# Autodesk Inventor assembly: ASY MSC 800 gills
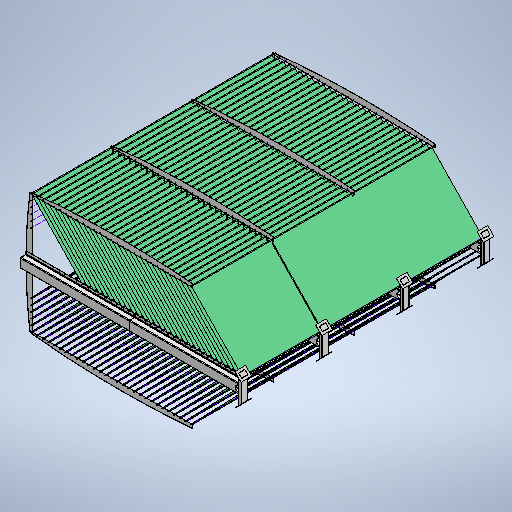
[picture p0: Inventor's stored thumbnail of the model, 512x512]
Saved by Autodesk Inventor 2025 (Build 290162010, 162A)
## iProperties
Created: 2024-08-31
Part Number: ASY MSC 800 gills
Document SubType Name: Assembly
Designer: pokla
Stock Number: ASY МОО 800 Жабры
Mass: 469810 g
Surface Area: 1.86943e+06 cm^2
Volume: 67870.7 cm^3
Density: 6.92212 g/cm^3
Author: pokla
## Documents named in this file (19)
- C:\Users\pokla\Documents\Inventor\Отстойник осветлитель\Manturovo_Se-clar-Gleb\ASY MSC 800 gills.iam
- C:\Users\pokla\Documents\Inventor\Отстойник осветлитель\Manturovo_Se-clar-Gleb\MSC 804 sheet gills.ipt
- C:\Users\pokla\Documents\Inventor\Отстойник осветлитель\Manturovo_Se-clar-Gleb\MSC 810 pillar gills.ipt
- C:\Users\pokla\Documents\Inventor\Отстойник осветлитель\Manturovo_Se-clar-Gleb\MSC 805 sheet gills.ipt
- C:\Users\pokla\Documents\Inventor\Отстойник осветлитель\Manturovo_Se-clar-Gleb\MSC 806 sheet gills.ipt
- C:\Users\pokla\Documents\Inventor\Отстойник осветлитель\Manturovo_Se-clar-Gleb\MSC 807 sheet gills.ipt
- C:\Users\pokla\Documents\Inventor\Отстойник осветлитель\Manturovo_Se-clar-Gleb\MSC 808 sheet gills.ipt
- C:\Users\pokla\Documents\Inventor\Отстойник осветлитель\Manturovo_Se-clar-Gleb\MSC 809 sheet gills.ipt
- C:\Users\pokla\Documents\Inventor\Отстойник осветлитель\Manturovo_Se-clar-Gleb\MSC 813 wall support gills.ipt
- C:\Users\pokla\Documents\Inventor\Отстойник осветлитель\Manturovo_Se-clar-Gleb\MSC 811 pillar gills.ipt
- C:\Users\pokla\Documents\Inventor\Отстойник осветлитель\Manturovo_Se-clar-Gleb\MSC 814 string for sheets gills.ipt
- C:\Users\pokla\Documents\Inventor\Отстойник осветлитель\Manturovo_Se-clar-Gleb\MSC 812 top support gills.ipt
- C:\Users\pokla\Documents\Inventor\Отстойник осветлитель\Manturovo_Se-clar-Gleb\MSC 803 sheet gills.ipt
- C:\Users\pokla\Documents\Inventor\Отстойник осветлитель\Manturovo_Se-clar-Gleb\ASY MSC 800.1 gills base.iam
- C:\Users\pokla\Documents\Inventor\Отстойник осветлитель\Manturovo_Se-clar-Gleb\MSC 805 sheet gills+.ipt
- C:\Users\pokla\Documents\Inventor\Отстойник осветлитель\Manturovo_Se-clar-Gleb\MSC 806 sheet gills+.ipt
- C:\Users\pokla\Documents\Inventor\Отстойник осветлитель\Manturovo_Se-clar-Gleb\MSC 807 sheet gills+.ipt
- C:\Users\pokla\Documents\Inventor\Отстойник осветлитель\Manturovo_Se-clar-Gleb\MSC 808 sheet gills+.ipt
- C:\Users\pokla\Documents\Inventor\Отстойник осветлитель\Manturovo_Se-clar-Gleb\MSC 809 sheet gills+.ipt
## Components (287 placed, 18 different names)
1. MSC 805 SHEET GILLS:1 — Angle:2, Tangent:8, Tangent:9, Flush:15, Flush:19, Rigid:42
2. MSC 806 SHEET GILLS:1 — Angle:3, Tangent:10, Tangent:11, Flush:15, Flush:16, Rigid:43
3. MSC 807 SHEET GILLS:1 — Angle:4, Tangent:12, Tangent:13, Flush:16, Flush:17, Rigid:45
4. MSC 808 SHEET GILLS:1 — Angle:5, Tangent:17, Tangent:18, Flush:17, Flush:18, Rigid:46
5. MSC 809 SHEET GILLS:1 — Angle:6, Tangent:19, Tangent:20, Flush:18, Rigid:47
6. MSC 814 STRING FOR SHEETS GILLS:1 — Rigid:40
7. MSC 805 SHEET GILLS+:1 — Rigid:42
8. MSC 806 SHEET GILLS+:1 — Rigid:43
9. MSC 807 SHEET GILLS+:1 — Rigid:45
10. MSC 808 SHEET GILLS+:1 — Rigid:46
11. MSC 809 SHEET GILLS+:1 — Rigid:47
12. MSC 814 STRING FOR SHEETS GILLS:2 — Rigid:24
13. MSC 814 STRING FOR SHEETS GILLS:3
14. MSC 814 STRING FOR SHEETS GILLS:4
15. MSC 814 STRING FOR SHEETS GILLS:5
16. MSC 814 STRING FOR SHEETS GILLS:6
17. MSC 814 STRING FOR SHEETS GILLS:7
18. MSC 814 STRING FOR SHEETS GILLS:8 — Rigid:12
19. MSC 803 SHEET GILLS:1 — Rigid:33, Angle:2, Angle:3, Angle:4, Angle:5, Angle:6, Tangent:14, Tangent:15, Tangent:16, Flush:19, Flush:24
20. MSC 804 SHEET GILLS:1 — Rigid:33
21. MSC 814 STRING FOR SHEETS GILLS:9 — Rotational:1
22. MSC 814 STRING FOR SHEETS GILLS:10 — Rotational:2, Tangent:23
23. MSC 814 STRING FOR SHEETS GILLS:11 — Rotational:3, Tangent:21, Tangent:22
24. MSC 803 SHEET GILLS:2 — Tangent:21, Tangent:23, Flush:24
25. MSC 804 SHEET GILLS:2 — Tangent:22
26. MSC 814 STRING FOR SHEETS GILLS:12
27. MSC 803 SHEET GILLS:3
28. MSC 804 SHEET GILLS:3
29. MSC 814 STRING FOR SHEETS GILLS:13
30. MSC 814 STRING FOR SHEETS GILLS:14
31. MSC 814 STRING FOR SHEETS GILLS:15
32. MSC 803 SHEET GILLS:4
33. MSC 804 SHEET GILLS:4
34. MSC 814 STRING FOR SHEETS GILLS:16
35. MSC 803 SHEET GILLS:5
36. MSC 804 SHEET GILLS:5
37. MSC 814 STRING FOR SHEETS GILLS:17
38. MSC 814 STRING FOR SHEETS GILLS:18
39. MSC 814 STRING FOR SHEETS GILLS:19
40. MSC 803 SHEET GILLS:6
41. MSC 804 SHEET GILLS:6
42. MSC 814 STRING FOR SHEETS GILLS:20
43. MSC 803 SHEET GILLS:7
44. MSC 804 SHEET GILLS:7
45. MSC 814 STRING FOR SHEETS GILLS:21
46. MSC 814 STRING FOR SHEETS GILLS:22
47. MSC 814 STRING FOR SHEETS GILLS:23
48. MSC 803 SHEET GILLS:8
49. MSC 804 SHEET GILLS:8
50. MSC 814 STRING FOR SHEETS GILLS:24
51. MSC 803 SHEET GILLS:9
52. MSC 804 SHEET GILLS:9
53. MSC 814 STRING FOR SHEETS GILLS:25
54. MSC 814 STRING FOR SHEETS GILLS:26
55. MSC 814 STRING FOR SHEETS GILLS:27
56. MSC 803 SHEET GILLS:10
57. MSC 804 SHEET GILLS:10
58. MSC 814 STRING FOR SHEETS GILLS:28
59. MSC 803 SHEET GILLS:11
60. MSC 804 SHEET GILLS:11
61. MSC 814 STRING FOR SHEETS GILLS:29
62. MSC 814 STRING FOR SHEETS GILLS:30
63. MSC 814 STRING FOR SHEETS GILLS:31
64. MSC 803 SHEET GILLS:12
65. MSC 804 SHEET GILLS:12
66. MSC 814 STRING FOR SHEETS GILLS:32
67. MSC 803 SHEET GILLS:13
68. MSC 804 SHEET GILLS:13
69. MSC 814 STRING FOR SHEETS GILLS:33
70. MSC 814 STRING FOR SHEETS GILLS:34
71. MSC 814 STRING FOR SHEETS GILLS:35
72. MSC 803 SHEET GILLS:14
73. MSC 804 SHEET GILLS:14
74. MSC 814 STRING FOR SHEETS GILLS:36
75. MSC 803 SHEET GILLS:15
76. MSC 804 SHEET GILLS:15
77. MSC 814 STRING FOR SHEETS GILLS:37
78. MSC 814 STRING FOR SHEETS GILLS:38
79. MSC 814 STRING FOR SHEETS GILLS:39
80. MSC 803 SHEET GILLS:16
81. MSC 804 SHEET GILLS:16
82. MSC 814 STRING FOR SHEETS GILLS:40
83. MSC 803 SHEET GILLS:17
84. MSC 804 SHEET GILLS:17
85. MSC 814 STRING FOR SHEETS GILLS:41
86. MSC 814 STRING FOR SHEETS GILLS:42
87. MSC 814 STRING FOR SHEETS GILLS:43
88. MSC 803 SHEET GILLS:18
89. MSC 804 SHEET GILLS:18
90. MSC 814 STRING FOR SHEETS GILLS:44
91. MSC 803 SHEET GILLS:19
92. MSC 804 SHEET GILLS:19
93. MSC 814 STRING FOR SHEETS GILLS:45
94. MSC 814 STRING FOR SHEETS GILLS:46
95. MSC 814 STRING FOR SHEETS GILLS:47
96. MSC 803 SHEET GILLS:20
97. MSC 804 SHEET GILLS:20
98. MSC 814 STRING FOR SHEETS GILLS:48
99. MSC 803 SHEET GILLS:21
100. MSC 804 SHEET GILLS:21
101. MSC 814 STRING FOR SHEETS GILLS:49
102. MSC 814 STRING FOR SHEETS GILLS:50
103. MSC 814 STRING FOR SHEETS GILLS:51
104. MSC 803 SHEET GILLS:22
105. MSC 804 SHEET GILLS:22
106. MSC 814 STRING FOR SHEETS GILLS:52
107. MSC 803 SHEET GILLS:23
108. MSC 804 SHEET GILLS:23
109. MSC 814 STRING FOR SHEETS GILLS:53
110. MSC 814 STRING FOR SHEETS GILLS:54
111. MSC 814 STRING FOR SHEETS GILLS:55
112. MSC 803 SHEET GILLS:24
113. MSC 804 SHEET GILLS:24
114. MSC 814 STRING FOR SHEETS GILLS:56
115. MSC 803 SHEET GILLS:25
116. MSC 804 SHEET GILLS:25
117. MSC 814 STRING FOR SHEETS GILLS:57
118. MSC 814 STRING FOR SHEETS GILLS:58
119. MSC 814 STRING FOR SHEETS GILLS:59
120. MSC 803 SHEET GILLS:26
121. MSC 804 SHEET GILLS:26
122. MSC 814 STRING FOR SHEETS GILLS:60
123. MSC 803 SHEET GILLS:27
124. MSC 804 SHEET GILLS:27
125. MSC 814 STRING FOR SHEETS GILLS:61
126. MSC 814 STRING FOR SHEETS GILLS:62
127. MSC 814 STRING FOR SHEETS GILLS:63
128. MSC 803 SHEET GILLS:28
129. MSC 804 SHEET GILLS:28
130. MSC 814 STRING FOR SHEETS GILLS:64
131. MSC 803 SHEET GILLS:29
132. MSC 804 SHEET GILLS:29
133. MSC 814 STRING FOR SHEETS GILLS:65
134. MSC 814 STRING FOR SHEETS GILLS:66
135. MSC 814 STRING FOR SHEETS GILLS:67
136. MSC 803 SHEET GILLS:30
137. MSC 804 SHEET GILLS:30
138. MSC 814 STRING FOR SHEETS GILLS:68
139. MSC 803 SHEET GILLS:31
140. MSC 804 SHEET GILLS:31
141. MSC 814 STRING FOR SHEETS GILLS:69
142. MSC 814 STRING FOR SHEETS GILLS:70
143. MSC 814 STRING FOR SHEETS GILLS:71
144. MSC 803 SHEET GILLS:32
145. MSC 804 SHEET GILLS:32
146. MSC 814 STRING FOR SHEETS GILLS:72
147. MSC 803 SHEET GILLS:33
148. MSC 804 SHEET GILLS:33
149. MSC 814 STRING FOR SHEETS GILLS:73
150. MSC 814 STRING FOR SHEETS GILLS:74
151. MSC 814 STRING FOR SHEETS GILLS:75
152. MSC 803 SHEET GILLS:34
153. MSC 804 SHEET GILLS:34
154. MSC 814 STRING FOR SHEETS GILLS:76
155. MSC 803 SHEET GILLS:35
156. MSC 804 SHEET GILLS:35
157. MSC 814 STRING FOR SHEETS GILLS:77
158. MSC 814 STRING FOR SHEETS GILLS:78
159. MSC 814 STRING FOR SHEETS GILLS:79
160. MSC 803 SHEET GILLS:36
161. MSC 804 SHEET GILLS:36
162. MSC 814 STRING FOR SHEETS GILLS:80
163. MSC 803 SHEET GILLS:37
164. MSC 804 SHEET GILLS:37
165. MSC 814 STRING FOR SHEETS GILLS:81
166. MSC 814 STRING FOR SHEETS GILLS:82
167. MSC 814 STRING FOR SHEETS GILLS:83
168. MSC 803 SHEET GILLS:38
169. MSC 804 SHEET GILLS:38
170. MSC 814 STRING FOR SHEETS GILLS:84
171. MSC 803 SHEET GILLS:39
172. MSC 804 SHEET GILLS:39
173. MSC 814 STRING FOR SHEETS GILLS:85
174. MSC 814 STRING FOR SHEETS GILLS:86
175. MSC 814 STRING FOR SHEETS GILLS:87
176. MSC 803 SHEET GILLS:40
177. MSC 804 SHEET GILLS:40
178. MSC 814 STRING FOR SHEETS GILLS:88
179. MSC 803 SHEET GILLS:41
180. MSC 804 SHEET GILLS:41
181. MSC 814 STRING FOR SHEETS GILLS:89
182. MSC 814 STRING FOR SHEETS GILLS:90
183. MSC 814 STRING FOR SHEETS GILLS:91
184. MSC 803 SHEET GILLS:42
185. MSC 804 SHEET GILLS:42
186. MSC 814 STRING FOR SHEETS GILLS:92
187. MSC 803 SHEET GILLS:43
188. MSC 804 SHEET GILLS:43
189. MSC 814 STRING FOR SHEETS GILLS:93
190. MSC 814 STRING FOR SHEETS GILLS:94
191. MSC 814 STRING FOR SHEETS GILLS:95
192. MSC 803 SHEET GILLS:44
193. MSC 804 SHEET GILLS:44
194. MSC 814 STRING FOR SHEETS GILLS:96
195. MSC 803 SHEET GILLS:45
196. MSC 804 SHEET GILLS:45
197. MSC 814 STRING FOR SHEETS GILLS:97
198. MSC 814 STRING FOR SHEETS GILLS:98
199. MSC 814 STRING FOR SHEETS GILLS:99
200. MSC 803 SHEET GILLS:46
201. MSC 804 SHEET GILLS:46
202. MSC 814 STRING FOR SHEETS GILLS:100
203. MSC 803 SHEET GILLS:47
204. MSC 804 SHEET GILLS:47
205. MSC 814 STRING FOR SHEETS GILLS:101
206. MSC 814 STRING FOR SHEETS GILLS:102
207. MSC 814 STRING FOR SHEETS GILLS:103
208. MSC 803 SHEET GILLS:48
209. MSC 804 SHEET GILLS:48
210. MSC 814 STRING FOR SHEETS GILLS:104
211. MSC 803 SHEET GILLS:49
212. MSC 804 SHEET GILLS:49
213. MSC 814 STRING FOR SHEETS GILLS:105
214. MSC 814 STRING FOR SHEETS GILLS:106
215. MSC 814 STRING FOR SHEETS GILLS:107
216. MSC 803 SHEET GILLS:50
217. MSC 804 SHEET GILLS:50
218. MSC 814 STRING FOR SHEETS GILLS:108
219. MSC 803 SHEET GILLS:51
220. MSC 804 SHEET GILLS:51
221. MSC 814 STRING FOR SHEETS GILLS:109
222. MSC 814 STRING FOR SHEETS GILLS:110
223. MSC 814 STRING FOR SHEETS GILLS:111
224. MSC 803 SHEET GILLS:52
225. MSC 804 SHEET GILLS:52
226. MSC 814 STRING FOR SHEETS GILLS:112
227. MSC 803 SHEET GILLS:53
228. MSC 804 SHEET GILLS:53
229. MSC 814 STRING FOR SHEETS GILLS:113
230. MSC 814 STRING FOR SHEETS GILLS:114
231. MSC 814 STRING FOR SHEETS GILLS:115
232. MSC 803 SHEET GILLS:54
233. MSC 804 SHEET GILLS:54
234. MSC 814 STRING FOR SHEETS GILLS:116
235. MSC 803 SHEET GILLS:55
236. MSC 804 SHEET GILLS:55
237. MSC 814 STRING FOR SHEETS GILLS:117
238. MSC 814 STRING FOR SHEETS GILLS:118
239. MSC 814 STRING FOR SHEETS GILLS:119
240. MSC 803 SHEET GILLS:56
241. MSC 804 SHEET GILLS:56
242. MSC 814 STRING FOR SHEETS GILLS:120
243. MSC 803 SHEET GILLS:57
244. MSC 804 SHEET GILLS:57
245. MSC 814 STRING FOR SHEETS GILLS:121
246. MSC 814 STRING FOR SHEETS GILLS:122
247. MSC 814 STRING FOR SHEETS GILLS:123
248. MSC 803 SHEET GILLS:58
249. MSC 804 SHEET GILLS:58
250. MSC 813 WALL SUPPORT GILLS:1 — Rigid:12, Rigid:30, Tangent:14, Tangent:15
251. MSC 812 TOP SUPPORT GILLS:1 — Rigid:28, Rigid:30, Tangent:8, Tangent:9, Tangent:10, Tangent:11, Tangent:12, Tangent:13, Tangent:17, Tangent:18, Tangent:19, Tangent:20, Rigid:40, Rigid:44
252. MSC 811 PILLAR GILLS:1 — Rigid:28, Rigid:29
253. MSC 812 TOP SUPPORT GILLS:2 — Rigid:24, Rigid:29, Rigid:31
254. MSC 813 WALL SUPPORT GILLS:2 — Rigid:31, Rotational:3
255. MSC 810 PILLAR GILLS:1 — Rotational:1, Rotational:2, Tangent:16
256. ASY MSC 800.1 gills base:1 [sub-assembly]
257. MSC 813 WALL SUPPORT GILLS:3
258. MSC 812 TOP SUPPORT GILLS:3
259. MSC 811 PILLAR GILLS:2
260. MSC 812 TOP SUPPORT GILLS:4
261. MSC 813 WALL SUPPORT GILLS:4
262. MSC 810 PILLAR GILLS:2
263. ASY MSC 800.1 gills base:2 [sub-assembly]
264. MSC 813 WALL SUPPORT GILLS:5
265. MSC 812 TOP SUPPORT GILLS:5
266. MSC 811 PILLAR GILLS:3
267. MSC 812 TOP SUPPORT GILLS:6
268. MSC 813 WALL SUPPORT GILLS:6
269. MSC 810 PILLAR GILLS:3
270. ASY MSC 800.1 gills base:3 [sub-assembly]
271. MSC 813 WALL SUPPORT GILLS:7
272. MSC 812 TOP SUPPORT GILLS:7
273. MSC 811 PILLAR GILLS:4 — Rotational:4
274. MSC 812 TOP SUPPORT GILLS:8
275. MSC 813 WALL SUPPORT GILLS:8
276. MSC 810 PILLAR GILLS:4
277. ASY MSC 800.1 gills base:4 [sub-assembly]
278. MSC 814 STRING FOR SHEETS GILLS:124 — Rotational:4
279. MSC 814 STRING FOR SHEETS GILLS:125
280. MSC 814 STRING FOR SHEETS GILLS:126
281. MSC 814 STRING FOR SHEETS GILLS:127
282. MSC 814 STRING FOR SHEETS GILLS:128
283. MSC 814 STRING FOR SHEETS GILLS:129 — Rigid:44
284. MSC 814 STRING FOR SHEETS GILLS:130
285. MSC 814 STRING FOR SHEETS GILLS:131
286. MSC 814 STRING FOR SHEETS GILLS:132
287. MSC 814 STRING FOR SHEETS GILLS:133
## Component patterns: (6 elements, first: MSC 814 STRING FOR SHEETS GILLS:2), (29 elements, first: MSC 814 STRING FOR SHEETS GILLS:8 + MSC 803 SHEET GILLS:1 + MSC 804 SHEET GILLS:1 + MSC 814 STRING FOR SHEETS GILLS:9 + MSC 814 STRING FOR SHEETS GILLS:10 + MSC 814 STRING FOR SHEETS GILLS:11 + MSC 803 SHEET GILLS:2 + MSC 804 SHEET GILLS:2), (4 elements, first: MSC 813 WALL SUPPORT GILLS:1 + MSC 812 TOP SUPPORT GILLS:1 + MSC 811 PILLAR GILLS:1 + MSC 812 TOP SUPPORT GILLS:2 + MSC 813 WALL SUPPORT GILLS:2 + MSC 810 PILLAR GILLS:1 + ASY MSC 800.1 gills base:1), (5 elements, first: MSC 814 STRING FOR SHEETS GILLS:124), (5 elements, first: MSC 814 STRING FOR SHEETS GILLS:129)
## Relationships (53: WeldJoint 16, Tangent 16, Flush 9, Angle 5, RevoluteJoint 4, Mate 3)
- [WeldJoint]: MSC 811 PILLAR GILLS:1 ↔ MSC 810 PILLAR GILLS:1
- [Flush]: MSC 810 PILLAR GILLS:1 ↔ ASY MSC 800.1 gills base:1
- [Mate]: MSC 810 PILLAR GILLS:1 ↔ ASY MSC 800.1 gills base:1
- [Flush] (5 mm): MSC 810 PILLAR GILLS:1 ↔ ASY MSC 800.1 gills base:1
- Rigid:12 [WeldJoint] (-5 mm): MSC 814 STRING FOR SHEETS GILLS:8 ↔ MSC 813 WALL SUPPORT GILLS:1
- [Mate]: ASY MSC 800.1 gills base:1
- [Mate]: ASY MSC 800.1 gills base:1
- [Flush]: ASY MSC 800.1 gills base:1
- Rigid:24 [WeldJoint] (-5 mm): MSC 814 STRING FOR SHEETS GILLS:2 ↔ MSC 812 TOP SUPPORT GILLS:2
- Rigid:28 [WeldJoint]: MSC 812 TOP SUPPORT GILLS:1 ↔ MSC 811 PILLAR GILLS:1
- Rigid:29 [WeldJoint]: MSC 811 PILLAR GILLS:1 ↔ MSC 812 TOP SUPPORT GILLS:2
- Rigid:30 [WeldJoint]: MSC 813 WALL SUPPORT GILLS:1 ↔ MSC 812 TOP SUPPORT GILLS:1
- Rigid:31 [WeldJoint]: MSC 812 TOP SUPPORT GILLS:2 ↔ MSC 813 WALL SUPPORT GILLS:2
- Rotational:1 [RevoluteJoint] (5 mm): MSC 814 STRING FOR SHEETS GILLS:9 ↔ MSC 810 PILLAR GILLS:1
- Rotational:2 [RevoluteJoint] (-5 mm): MSC 814 STRING FOR SHEETS GILLS:10 ↔ MSC 810 PILLAR GILLS:1
- Rigid:33 [WeldJoint] (-10 mm): MSC 803 SHEET GILLS:1 ↔ MSC 804 SHEET GILLS:1
- Angle:2 (0 deg): MSC 805 SHEET GILLS:1 ↔ MSC 803 SHEET GILLS:1
- Angle:3 (0 deg): MSC 806 SHEET GILLS:1 ↔ MSC 803 SHEET GILLS:1
- Angle:4 (0 deg): MSC 807 SHEET GILLS:1 ↔ MSC 803 SHEET GILLS:1
- Angle:5 (0 deg): MSC 808 SHEET GILLS:1 ↔ MSC 803 SHEET GILLS:1
- Angle:6 (0 deg): MSC 809 SHEET GILLS:1 ↔ MSC 803 SHEET GILLS:1
- Tangent:8: MSC 805 SHEET GILLS:1 ↔ MSC 812 TOP SUPPORT GILLS:1
- Tangent:9: MSC 805 SHEET GILLS:1 ↔ MSC 812 TOP SUPPORT GILLS:1
- Tangent:10: MSC 806 SHEET GILLS:1 ↔ MSC 812 TOP SUPPORT GILLS:1
- Tangent:11: MSC 806 SHEET GILLS:1 ↔ MSC 812 TOP SUPPORT GILLS:1
- Tangent:12: MSC 807 SHEET GILLS:1 ↔ MSC 812 TOP SUPPORT GILLS:1
- Tangent:13: MSC 807 SHEET GILLS:1 ↔ MSC 812 TOP SUPPORT GILLS:1
- Tangent:14: MSC 803 SHEET GILLS:1 ↔ MSC 813 WALL SUPPORT GILLS:1
- Tangent:15: MSC 803 SHEET GILLS:1 ↔ MSC 813 WALL SUPPORT GILLS:1
- Tangent:16: MSC 803 SHEET GILLS:1 ↔ MSC 810 PILLAR GILLS:1
- Tangent:17: MSC 808 SHEET GILLS:1 ↔ MSC 812 TOP SUPPORT GILLS:1
- Tangent:18: MSC 808 SHEET GILLS:1 ↔ MSC 812 TOP SUPPORT GILLS:1
- Tangent:19: MSC 809 SHEET GILLS:1 ↔ MSC 812 TOP SUPPORT GILLS:1
- Tangent:20: MSC 809 SHEET GILLS:1 ↔ MSC 812 TOP SUPPORT GILLS:1
- Flush:15: MSC 805 SHEET GILLS:1 ↔ MSC 806 SHEET GILLS:1
- Flush:16: MSC 806 SHEET GILLS:1 ↔ MSC 807 SHEET GILLS:1
- Flush:17: MSC 807 SHEET GILLS:1 ↔ MSC 808 SHEET GILLS:1
- Flush:18: MSC 808 SHEET GILLS:1 ↔ MSC 809 SHEET GILLS:1
- Flush:19: MSC 805 SHEET GILLS:1 ↔ MSC 803 SHEET GILLS:1
- Rigid:40 [WeldJoint] (5 mm): MSC 814 STRING FOR SHEETS GILLS:1 ↔ MSC 812 TOP SUPPORT GILLS:1
- Rotational:3 [RevoluteJoint] (-5 mm): MSC 814 STRING FOR SHEETS GILLS:11 ↔ MSC 813 WALL SUPPORT GILLS:2
- [WeldJoint] (-10 mm): MSC 803 SHEET GILLS:2 ↔ MSC 804 SHEET GILLS:2
- Tangent:21: MSC 814 STRING FOR SHEETS GILLS:11 ↔ MSC 803 SHEET GILLS:2
- Tangent:22: MSC 814 STRING FOR SHEETS GILLS:11 ↔ MSC 804 SHEET GILLS:2
- Tangent:23: MSC 814 STRING FOR SHEETS GILLS:10 ↔ MSC 803 SHEET GILLS:2
- Flush:24: MSC 803 SHEET GILLS:1 ↔ MSC 803 SHEET GILLS:2
- Rigid:42 [WeldJoint] (-10 mm): MSC 805 SHEET GILLS:1 ↔ MSC 805 SHEET GILLS+:1
- Rotational:4 [RevoluteJoint] (22 mm): MSC 811 PILLAR GILLS:4 ↔ MSC 814 STRING FOR SHEETS GILLS:124
- Rigid:43 [WeldJoint] (-10 mm): MSC 806 SHEET GILLS:1 ↔ MSC 806 SHEET GILLS+:1
- Rigid:44 [WeldJoint] (5 mm): MSC 812 TOP SUPPORT GILLS:1 ↔ MSC 814 STRING FOR SHEETS GILLS:129
- Rigid:45 [WeldJoint] (-10 mm): MSC 807 SHEET GILLS:1 ↔ MSC 807 SHEET GILLS+:1
- Rigid:46 [WeldJoint] (-10 mm): MSC 808 SHEET GILLS:1 ↔ MSC 808 SHEET GILLS+:1
- Rigid:47 [WeldJoint] (-10 mm): MSC 809 SHEET GILLS:1 ↔ MSC 809 SHEET GILLS+:1
